# Autodesk Inventor assembly: CL6-200
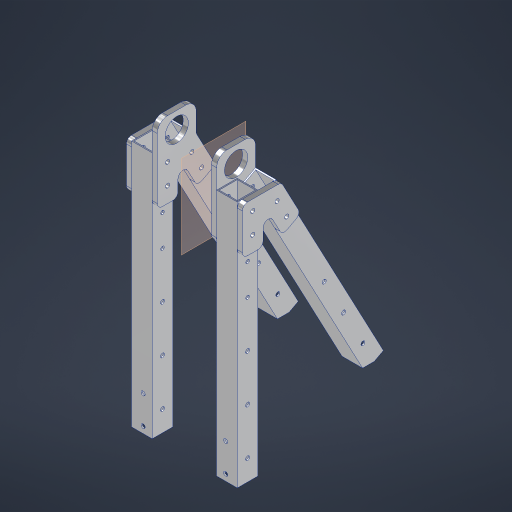
[picture p0: Inventor's stored thumbnail of the model, 512x512]
Saved by Autodesk Inventor 2023.4 (Build 274418000, 418)
## iProperties
Created: 2025-02-04
Part Number: CL6-200
Document SubType Name: Assembly
Designer: brand
Mass: 705.105 g
Surface Area: 2600.93 cm^2
Volume: 261.15 cm^3
Density: 2.7 g/cm^3
Author: brand
## Documents named in this file (5)
- C:\Users\brand\OneDrive\Documents\GitHub\robotics 23\2025-ReefScape---CAD\Climber\CL6\CL6-200.iam
- C:\Users\brand\OneDrive\Documents\GitHub\robotics 23\2025-ReefScape---CAD\Climber\CL4\CL4-002.ipt
- C:\Users\brand\OneDrive\Documents\GitHub\robotics 23\2025-ReefScape---CAD\Climber\CL4\CL4-007.ipt
- C:\Users\brand\OneDrive\Documents\GitHub\robotics 23\2025-ReefScape---CAD\Climber\CL4\CL4-009.ipt
- C:\Users\brand\OneDrive\Documents\GitHub\robotics 23\2025-ReefScape---CAD\Climber\CL4\CL4-010.ipt
## Components (8 placed, 4 different names)
1. CL4-002:1 — Flush:2, Flush:3, Insert:13, Insert:14
2. CL4-002:2 — Flush:2, Insert:5, Insert:6, Insert:11, Flush:3
3. CL4-007:1 — Insert:7, Insert:8, Insert:12
4. CL4-007:2 — Insert:3, Insert:4, Insert:10
5. CL4-009:1 — Insert:3, Insert:4, Insert:14
6. CL4-009:2 — Insert:5, Insert:6, Insert:7, Insert:8
7. CL4-010:1 — Insert:10, Symmetry:1, Mate:1, Insert:13
8. CL4-010:2 — Insert:11, Insert:12, Symmetry:1, Mate:1
## Relationships (15: Insert 11, Flush 2, Symmetry 1, Mate 1)
- Flush:2: CL4-002:1 ↔ CL4-002:2
- Insert:3: CL4-007:2 ↔ CL4-009:1
- Insert:4: CL4-007:2 ↔ CL4-009:1
- Insert:5: CL4-002:2 ↔ CL4-009:2
- Insert:6: CL4-002:2 ↔ CL4-009:2
- Insert:7: CL4-007:1 ↔ CL4-009:2
- Insert:8: CL4-007:1 ↔ CL4-009:2
- Insert:10: CL4-007:2 ↔ CL4-010:1
- Insert:11: CL4-002:2 ↔ CL4-010:2
- Insert:12: CL4-007:1 ↔ CL4-010:2
- Symmetry:1: CL4-010:1 ↔ CL4-010:2
- Mate:1 (66.675 mm): CL4-010:1 ↔ CL4-010:2
- Flush:3: CL4-002:1 ↔ CL4-002:2
- Insert:13: CL4-002:1 ↔ CL4-010:1
- Insert:14: CL4-002:1 ↔ CL4-009:1
